# Autodesk Inventor assembly: EFOI-10
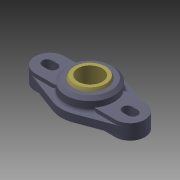
[picture p0: Inventor's stored thumbnail of the model, 180x180]
Saved by Autodesk Inventor 2013 (Build 170138000, 138)
## iProperties
Category: Plastic Bearings
Company: Autodesk, Inc.
Created: 2012-11-28
Part Number: EFOI-10
Document SubType Name: Assembly
Project: FIRST
Catalog Web Link: http://www.igus.com/wpck/default.aspx?pagenr=2504
Description: Flanged spherical bearing
Vendor: igus
Title: Flanged Spherical Bearing
Author: Autodesk, Inc.
## Documents named in this file (3)
- C:\Data Folder\FIRST 2013\FIRST KOP\Parts\Plastic Bearings\PB_Bearing_EFOI-10.iam
- C:\Data Folder\FIRST 2013\FIRST KOP\Parts\Plastic Bearings\EFOI-10_Housing.ipt
- C:\Data Folder\FIRST 2013\FIRST KOP\Parts\Plastic Bearings\EFOI-10_Spherical Bearing.ipt
## Components (2 placed, 2 different names)
1. EFOI-10_Housing:1 — Mate:1
2. EFOI-10_Spherical Bearing:1 — Mate:1
## Relationships (1: Mate 1)
- Mate:1: EFOI-10_Housing:1 ↔ EFOI-10_Spherical Bearing:1
